# Autodesk Inventor assembly: Sun
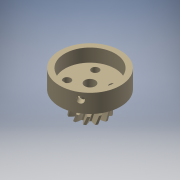
[picture p0: Inventor's stored thumbnail of the model, 180x180]
Saved by Autodesk Inventor 2019.1 (Build 231200000, 200)
## iProperties
Created: 2019-01-08
Part Number: Sun
Material: Generisch
Document SubType Name: Assembly
Designer: JochenAlt
Author: JochenAlt
## Documents named in this file (3)
- D:\Projects\Ondine\CAD\PlanetaryGear2\Sun.iam
- D:\Projects\Ondine\CAD\PlanetaryGear2\PlanetaryGearConstruction\Stirnzahnrad2-21.ipt
- D:\Projects\Ondine\CAD\PlanetaryGear2\Input.ipt
## Components (2 placed, 2 different names)
1. Sun:1 — Passend:1, Passend:2
2. Input:1 — Passend:1, Passend:2
## Relationships (2: Mate 2)
- Passend:1 [Mate]: Sun:1 ↔ Input:1
- Passend:2 [Mate]: Sun:1 ↔ Input:1
